# Autodesk Inventor assembly: PCB_Components
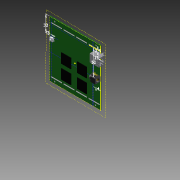
[picture p0: Inventor's stored thumbnail of the model, 180x180]
Saved by Autodesk Inventor 2015 SP1 (Build 190203100, 203)
## iProperties
Created: 2015-01-22
Part Number: PCB_Components
Document SubType Name: Assembly
Designer: Patrick
Author: Patrick
## Documents named in this file (5)
- C:\Users\Patrick\CAD\Spin3 Enclosure\PCB_Components.iam
- C:\Users\Patrick\CAD\Spin3 Enclosure\PCB.ipt
- C:\Users\Patrick\CAD\Spin3 Enclosure\Imported Components\DCJack_RAPC722X\DCJack_RAPC722X.ipt
- C:\Users\Patrick\CAD\Spin3 Enclosure\Imported Components\Pushbutton_KT11P2SM\Pushbutton_KT11P2SM.ipt
- C:\Users\Patrick\CAD\Spin3 Enclosure\Imported Components\EthernetJack_722310881lf\EthernetJack_722310881lf.ipt
## Components (4 placed, 4 different names)
1. PCB:1 — Mate:4, Mate:5, Mate:6, Mate:7, Mate:8, Mate:9, Mate:10, Mate:11
2. DCJack_RAPC722X:1 — Mate:4, Mate:5, Mate:6
3. Pushbutton_KT11P2SM:1 — Mate:7, Mate:8, Mate:9
4. EthernetJack_722310881lf:1 — Mate:10, Mate:11
## Relationships (8: Mate 8)
- Mate:4: PCB:1 ↔ DCJack_RAPC722X:1
- Mate:5: PCB:1 ↔ DCJack_RAPC722X:1
- Mate:6: PCB:1 ↔ DCJack_RAPC722X:1
- Mate:7: PCB:1 ↔ Pushbutton_KT11P2SM:1
- Mate:8: PCB:1 ↔ Pushbutton_KT11P2SM:1
- Mate:9: PCB:1 ↔ Pushbutton_KT11P2SM:1
- Mate:10: PCB:1 ↔ EthernetJack_722310881lf:1
- Mate:11: PCB:1 ↔ EthernetJack_722310881lf:1
